# Autodesk Inventor assembly: oil_tank_Assembly
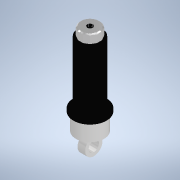
[picture p0: Inventor's stored thumbnail of the model, 180x180]
Saved by Autodesk Inventor 2020.2 (Build 242310000, 310)
## iProperties
Created: 2019-12-06
Part Number: oil_tank_Assembly
Document SubType Name: Assembly
Designer: axelj
Author: axelj
## Documents named in this file (5)
- C:\Users\axelj\OneDrive\Documentos\GitHub\autobot\robot_model\oil_tank_Assembly.iam
- C:\Users\axelj\OneDrive\Documentos\GitHub\autobot\robot_model\RCT-T005_Piston(Deposito_deAceite).ipt
- C:\Users\axelj\OneDrive\Documentos\GitHub\autobot\robot_model\RCT-T005_Elemento_externo.ipt
- C:\Users\axelj\OneDrive\Documentos\GitHub\autobot\robot_model\RCT-T005_Cubierta.ipt
- C:\Users\axelj\OneDrive\Documentos\GitHub\autobot\robot_model\RCT-T005_Conexion_inferior.ipt
## Components (4 placed, 4 different names)
1. RCT-T005_Piston(Deposito_deAceite):1 — Rígido:1, Rígido:2, De rotación:1
2. RCT-T005_Elemento_externo:1 — Rígido:2
3. RCT-T005_Cubierta:1 — De rotación:1
4. RCT-T005_Conexion_inferior:1 — Rígido:1
## Relationships (3: WeldJoint 2, RevoluteJoint 1)
- Rígido:1 [WeldJoint] (-0.0254 mm): RCT-T005_Piston(Deposito_deAceite):1 ↔ RCT-T005_Conexion_inferior:1
- Rígido:2 [WeldJoint]: RCT-T005_Piston(Deposito_deAceite):1 ↔ RCT-T005_Elemento_externo:1
- De rotación:1 [RevoluteJoint] (0.0254 mm): RCT-T005_Piston(Deposito_deAceite):1 ↔ RCT-T005_Cubierta:1
